# Autodesk Inventor assembly: 276-2177
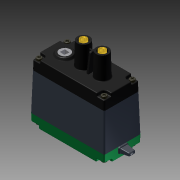
[picture p0: Inventor's stored thumbnail of the model, 180x180]
Saved by Autodesk Inventor 2014 SP1 (Build 180222100, 222)
## iProperties
Category: Motors
Company: Autodesk Inc.
Created: 2011-12-15
Part Number: 276-2177
Document SubType Name: Assembly
Designer: Autodesk Inc.
Catalog Web Link: http://www.vexrobotics.com/276-2177.html
Vendor: IFI
Description: 2-wire motor 393
Mass: 30.242 g
Surface Area: 365.411 cm^2
Volume: 30.242 cm^3
Density: 1 g/cm^3
Author: Autodesk Inc.
## Documents named in this file (21)
- C:\Users\Moses\Documents\GitHub\frc2014CAD\2012\Repackaged_Team_3061_Yr2012_Ball_Shooter\Motors_IFI_276-2177.iam
- C:\Users\Moses\Documents\GitHub\frc2014CAD\2012\Repackaged_Team_3061_Yr2012_Ball_Shooter\SPPM206-0150BO.ipt
- C:\Users\Moses\Documents\GitHub\frc2014CAD\2012\Repackaged_Team_3061_Yr2012_Ball_Shooter\SPPM204-0050BO.ipt
- C:\Users\Moses\Documents\GitHub\frc2014CAD\2012\Repackaged_Team_3061_Yr2012_Ball_Shooter\276-2177-002 Rev1.ipt
- C:\Users\Moses\Documents\GitHub\frc2014CAD\2012\Repackaged_Team_3061_Yr2012_Ball_Shooter\276-2177-008 Rev1.ipt
- C:\Users\Moses\Documents\GitHub\frc2014CAD\2012\Repackaged_Team_3061_Yr2012_Ball_Shooter\276-2177-010 Rev1.ipt
- C:\Users\Moses\Documents\GitHub\frc2014CAD\2012\Repackaged_Team_3061_Yr2012_Ball_Shooter\276-2177-001 Rev1.ipt
- C:\Users\Moses\Documents\GitHub\frc2014CAD\2012\Repackaged_Team_3061_Yr2012_Ball_Shooter\276-2177-012 Rev1.ipt
- C:\Users\Moses\Documents\GitHub\frc2014CAD\2012\Repackaged_Team_3061_Yr2012_Ball_Shooter\276-2177-018 Rev1.ipt
- C:\Users\Moses\Documents\GitHub\frc2014CAD\2012\Repackaged_Team_3061_Yr2012_Ball_Shooter\276-2177-014 Rev1.ipt
- C:\Users\Moses\Documents\GitHub\frc2014CAD\2012\Repackaged_Team_3061_Yr2012_Ball_Shooter\276-2177-019 Rev1.ipt
- C:\Users\Moses\Documents\GitHub\frc2014CAD\2012\Repackaged_Team_3061_Yr2012_Ball_Shooter\276-2177-017 Rev1.ipt
- C:\Users\Moses\Documents\GitHub\frc2014CAD\2012\Repackaged_Team_3061_Yr2012_Ball_Shooter\276-2177-004 Rev1.ipt
- C:\Users\Moses\Documents\GitHub\frc2014CAD\2012\Repackaged_Team_3061_Yr2012_Ball_Shooter\FS130-FT-21100.ipt
- C:\Users\Moses\Documents\GitHub\frc2014CAD\2012\Repackaged_Team_3061_Yr2012_Ball_Shooter\276-2177-006 Rev1.ipt
- C:\Users\Moses\Documents\GitHub\frc2014CAD\2012\Repackaged_Team_3061_Yr2012_Ball_Shooter\276-2177-009 Rev1.ipt
- C:\Users\Moses\Documents\GitHub\frc2014CAD\2012\Repackaged_Team_3061_Yr2012_Ball_Shooter\276-2177-011 Rev1.ipt
- C:\Users\Moses\Documents\GitHub\frc2014CAD\2012\Repackaged_Team_3061_Yr2012_Ball_Shooter\276-2177-007 Rev1_276-2177-007a.ipt
- C:\Users\Moses\Documents\GitHub\frc2014CAD\2012\Repackaged_Team_3061_Yr2012_Ball_Shooter\276-2177-013 Rev1.ipt
- C:\Users\Moses\Documents\GitHub\frc2014CAD\2012\Repackaged_Team_3061_Yr2012_Ball_Shooter\276-2177-003 Rev1.ipt
- C:\Users\Moses\Documents\GitHub\frc2014CAD\2012\Repackaged_Team_3061_Yr2012_Ball_Shooter\276-2177-005 Rev1.ipt
## Components (29 placed, 20 different names)
1. SPPM206-0150BO:1 — Insert:7
2. SPPM206-0150BO:2 — Insert:4
3. SPPM204-0050BO:1 — Insert:15
4. 276-2177-002 Rev1:1 — Mate:1, Mate:2, Flush:1, Mate:3, Mate:4, Mate:5, Insert:13, Flush:2, Flush:3, Flush:4, Insert:15, Insert:16, Mate:7, Flush:7, Flush:8, Mate:10, Flush:9, Mate:12, Flush:11, Flush:12, Mate:13
5. SPPM206-0150BO:3 — Insert:5, Mate:1
6. 276-2177-008 Rev1:1 — Insert:3, Insert:8
7. 276-2177-010 Rev1:1 — Mate:9, Mate:10, Flush:10
8. 276-2177-001 Rev1:1 — Mate:3, Mate:4, Mate:5, Insert:9, Insert:10, Insert:11, Insert:12
9. 276-2177-012 Rev1:1 — Insert:13
10. 276-2177-018 Rev1:1 — Flush:11, Flush:12, Mate:13
11. 276-2177-014 Rev1:1 — Insert:14, Flush:2, Flush:3, Flush:4, Flush:5
12. 276-2177-019 Rev1:1 — Insert:2
13. 276-2177-017 Rev1:1
14. SPPM206-0150BO:4 — Insert:9
15. 276-2177-004 Rev1:1 — Flush:6, Mate:6
16. SPPM206-0150BO:5 — Insert:10
17. 276-2177-019 Rev1:2 — Insert:1
18. SPPM204-0050BO:2 — Insert:16
19. FS130-FT-21100:1 — Insert:14, Flush:5, Flush:6, Mate:6
20. 276-2177-006 Rev1:1 — Mate:9, Flush:8, Flush:10
21. 276-2177-009 Rev1:1 — Mate:11, Mate:12
22. 276-2177-011 Rev1:1 — Mate:7, Mate:8
23. 276-2177-007 Rev1_276-2177-007a:1 — Mate:11, Flush:9
24. 276-2177-013 Rev1:1 — Insert:8
25. SPPM206-0150BO:6 — Insert:11
26. 276-2177-003 Rev1:1 — Insert:1, Insert:2, Insert:3, Insert:4, Insert:5, Insert:6, Insert:7, Mate:2, Flush:1
27. SPPM206-0150BO:7 — Insert:12
28. 276-2177-005 Rev1:1 — Mate:8, Flush:7
29. SPPM206-0150BO:8 — Insert:6
## Relationships (41: Insert 16, Mate 13, Flush 12)
- Insert:1 (-0.635 mm): 276-2177-019 Rev1:2 ↔ 276-2177-003 Rev1:1
- Insert:2 (-0.635 mm): 276-2177-019 Rev1:1 ↔ 276-2177-003 Rev1:1
- Insert:3: 276-2177-008 Rev1:1 ↔ 276-2177-003 Rev1:1
- Insert:4: SPPM206-0150BO:2 ↔ 276-2177-003 Rev1:1
- Insert:5: SPPM206-0150BO:3 ↔ 276-2177-003 Rev1:1
- Insert:6: 276-2177-003 Rev1:1 ↔ SPPM206-0150BO:8
- Insert:7: SPPM206-0150BO:1 ↔ 276-2177-003 Rev1:1
- Mate:1: 276-2177-002 Rev1:1 ↔ SPPM206-0150BO:3
- Insert:8 (-2.9972 mm): 276-2177-008 Rev1:1 ↔ 276-2177-013 Rev1:1
- Mate:2: 276-2177-002 Rev1:1 ↔ 276-2177-003 Rev1:1
- Flush:1: 276-2177-002 Rev1:1 ↔ 276-2177-003 Rev1:1
- Mate:3: 276-2177-002 Rev1:1 ↔ 276-2177-001 Rev1:1
- Mate:4: 276-2177-002 Rev1:1 ↔ 276-2177-001 Rev1:1
- Mate:5: 276-2177-002 Rev1:1 ↔ 276-2177-001 Rev1:1
- Insert:9: 276-2177-001 Rev1:1 ↔ SPPM206-0150BO:4
- Insert:10: 276-2177-001 Rev1:1 ↔ SPPM206-0150BO:5
- Insert:11: 276-2177-001 Rev1:1 ↔ SPPM206-0150BO:6
- Insert:12: 276-2177-001 Rev1:1 ↔ SPPM206-0150BO:7
- Insert:13: 276-2177-002 Rev1:1 ↔ 276-2177-012 Rev1:1
- Insert:14 (-1.0922 mm): 276-2177-014 Rev1:1 ↔ FS130-FT-21100:1
- Flush:2 (0.8382 mm): 276-2177-002 Rev1:1 ↔ 276-2177-014 Rev1:1
- Flush:3 (1.3462 mm): 276-2177-002 Rev1:1 ↔ 276-2177-014 Rev1:1
- Flush:4 (-3.556 mm): 276-2177-002 Rev1:1 ↔ 276-2177-014 Rev1:1
- Flush:5: 276-2177-014 Rev1:1 ↔ FS130-FT-21100:1
- Insert:15: SPPM204-0050BO:1 ↔ 276-2177-002 Rev1:1
- Insert:16: 276-2177-002 Rev1:1 ↔ SPPM204-0050BO:2
- Flush:6 (-0.4064 mm): 276-2177-004 Rev1:1 ↔ FS130-FT-21100:1
- Mate:6: 276-2177-004 Rev1:1 ↔ FS130-FT-21100:1
- Mate:7: 276-2177-002 Rev1:1 ↔ 276-2177-011 Rev1:1
- Mate:8: 276-2177-011 Rev1:1 ↔ 276-2177-005 Rev1:1
- Flush:7 (-2.3876 mm): 276-2177-002 Rev1:1 ↔ 276-2177-005 Rev1:1
- Mate:9: 276-2177-010 Rev1:1 ↔ 276-2177-006 Rev1:1
- Flush:8 (0.7112 mm): 276-2177-002 Rev1:1 ↔ 276-2177-006 Rev1:1
- Mate:10: 276-2177-002 Rev1:1 ↔ 276-2177-010 Rev1:1
- Mate:11: 276-2177-009 Rev1:1 ↔ 276-2177-007 Rev1_276-2177-007a:1
- Flush:9 (5.7404 mm): 276-2177-002 Rev1:1 ↔ 276-2177-007 Rev1_276-2177-007a:1
- Mate:12: 276-2177-002 Rev1:1 ↔ 276-2177-009 Rev1:1
- Flush:10 (-2.8194 mm): 276-2177-010 Rev1:1 ↔ 276-2177-006 Rev1:1
- Flush:11 (-3.2004 mm): 276-2177-002 Rev1:1 ↔ 276-2177-018 Rev1:1
- Flush:12 (-9.4996 mm): 276-2177-002 Rev1:1 ↔ 276-2177-018 Rev1:1
- Mate:13 (0.7874 mm): 276-2177-002 Rev1:1 ↔ 276-2177-018 Rev1:1
